# Autodesk Inventor assembly: HbBatteryCase
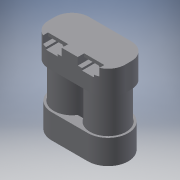
[picture p0: Inventor's stored thumbnail of the model, 180x180]
Saved by Autodesk Inventor 2018.1 (Build 221171000, 171)
## iProperties
Created: 2017-09-02
Part Number: HbBatteryCase
Material: 一般
Document SubType Name: Assembly
Designer: sktom
Author: sktom
## Documents named in this file (4)
- D:\CloudStrage\OneDrive\CAD\MAJ\hackberry\HACKberry-hardware\3D_69%inlength\Inventor\HbBatteryCase\HbBatteryCase.iam
- D:\CloudStrage\OneDrive\CAD\MAJ\hackberry\HACKberry-hardware\3D_69%inlength\Inventor\HbBatteryCase\CaseBottom_CR123A.ipt
- D:\CloudStrage\OneDrive\CAD\MAJ\hackberry\HACKberry-hardware\3D_69%inlength\Inventor\HbBatteryCase\CR123A.ipt
- D:\CloudStrage\OneDrive\CAD\MAJ\hackberry\HACKberry-hardware\3D_69%inlength\Inventor\HbBatteryCase\CaseTop_CR123A.ipt
## Components (4 placed, 3 different names)
1. CaseBottom_CR123A:1 — 挿入:1, 挿入:2
2. CR123A:1 — 挿入:2, 挿入:3
3. CR123A:2 — 挿入:1, 挿入:4
4. CaseTop_CR123A:1 — 挿入:3, 挿入:4
## Relationships (4: Insert 4)
- 挿入:1 [Insert]: CaseBottom_CR123A:1 ↔ CR123A:2
- 挿入:2 [Insert]: CaseBottom_CR123A:1 ↔ CR123A:1
- 挿入:3 [Insert]: CR123A:1 ↔ CaseTop_CR123A:1
- 挿入:4 [Insert]: CR123A:2 ↔ CaseTop_CR123A:1
